# Autodesk Inventor assembly: mearm 期末組合
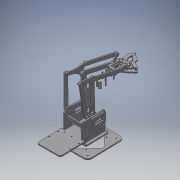
[picture p0: Inventor's stored thumbnail of the model, 180x180]
Saved by Autodesk Inventor 2019 (Build 230136000, 136)
## iProperties
Created: 2022-01-10
Part Number: mearm 期末組合
Material: 一般
Document SubType Name: Assembly
Designer: 10617
Author: 10617
## Documents named in this file (31)
- E:\cad2021\data\tmp\cad2021_hw\downloads\meARM\meARM_Inventor\HW1_mearm零組件\HW1_mearm組合.iam
- E:\cad2021\data\tmp\cad2021_hw\downloads\meARM\meARM_Inventor\HW1_mearm零組件\1.ipt
- E:\cad2021\data\tmp\cad2021_hw\downloads\meARM\meARM_Inventor\HW1_mearm零組件\2.ipt
- E:\cad2021\data\tmp\cad2021_hw\downloads\meARM\meARM_Inventor\HW1_mearm零組件\3.ipt
- E:\cad2021\data\tmp\cad2021_hw\downloads\meARM\meARM_Inventor\HW1_mearm零組件\4.ipt
- E:\cad2021\data\tmp\cad2021_hw\downloads\meARM\meARM_Inventor\HW1_mearm零組件\5.ipt
- E:\cad2021\data\tmp\cad2021_hw\downloads\meARM\meARM_Inventor\HW1_mearm零組件\6.ipt
- E:\cad2021\data\tmp\cad2021_hw\downloads\meARM\meARM_Inventor\HW1_mearm零組件\7.ipt
- E:\cad2021\data\tmp\cad2021_hw\downloads\meARM\meARM_Inventor\HW1_mearm零組件\8.ipt
- E:\cad2021\data\tmp\cad2021_hw\downloads\meARM\meARM_Inventor\HW1_mearm零組件\9.ipt
- E:\cad2021\data\tmp\cad2021_hw\downloads\meARM\meARM_Inventor\HW1_mearm零組件\10.ipt
- E:\cad2021\data\tmp\cad2021_hw\downloads\meARM\meARM_Inventor\HW1_mearm零組件\11.ipt
- E:\cad2021\data\tmp\cad2021_hw\downloads\meARM\meARM_Inventor\HW1_mearm零組件\12.ipt
- E:\cad2021\data\tmp\cad2021_hw\downloads\meARM\meARM_Inventor\HW1_mearm零組件\13.ipt
- E:\cad2021\data\tmp\cad2021_hw\downloads\meARM\meARM_Inventor\HW1_mearm零組件\14.ipt
- E:\cad2021\data\tmp\cad2021_hw\downloads\meARM\meARM_Inventor\HW1_mearm零組件\15.ipt
- E:\cad2021\data\tmp\cad2021_hw\downloads\meARM\meARM_Inventor\HW1_mearm零組件\16.ipt
- E:\cad2021\data\tmp\cad2021_hw\downloads\meARM\meARM_Inventor\HW1_mearm零組件\17.ipt
- E:\cad2021\data\tmp\cad2021_hw\downloads\meARM\meARM_Inventor\HW1_mearm零組件\18.ipt
- E:\cad2021\data\tmp\cad2021_hw\downloads\meARM\meARM_Inventor\HW1_mearm零組件\19.ipt
- E:\cad2021\data\tmp\cad2021_hw\downloads\meARM\meARM_Inventor\HW1_mearm零組件\20.ipt
- E:\cad2021\data\tmp\cad2021_hw\downloads\meARM\meARM_Inventor\HW1_mearm零組件\21.ipt
- E:\cad2021\data\tmp\cad2021_hw\downloads\meARM\meARM_Inventor\HW1_mearm零組件\22.ipt
- E:\cad2021\data\tmp\cad2021_hw\downloads\meARM\meARM_Inventor\HW1_mearm零組件\24.ipt
- E:\cad2021\data\tmp\cad2021_hw\downloads\meARM\meARM_Inventor\HW1_mearm零組件\25.ipt
- E:\cad2021\data\tmp\cad2021_hw\downloads\meARM\meARM_Inventor\HW1_mearm零組件\26.ipt
- E:\cad2021\data\tmp\cad2021_hw\downloads\meARM\meARM_Inventor\HW1_mearm零組件\27.ipt
- E:\cad2021\data\tmp\cad2021_hw\downloads\meARM\meARM_Inventor\HW1_mearm零組件\齒輪.ipt
- E:\cad2021\data\tmp\cad2021_hw\downloads\meARM\meARM_Inventor\HW1_mearm零組件\齒輪2.ipt
- E:\cad2021\data\tmp\cad2021_hw\downloads\meARM\meARM_Inventor\HW1_mearm零組件\23.ipt
- E:\cad2021\data\tmp\cad2021_hw\downloads\meARM\meARM_Inventor\HW1_mearm零組件\軸.ipt
## Components (48 placed, 30 different names)
1. 1:1 — 貼合:30, 貼合:31, 貼合:32, 貼合:42, 貼合:46, 貼合:47
2. 2:1 — 貼合:33, 貼合:34, 貼合:35, 貼合:36, 貼合:37, 貼合:41
3. 3:1 — 貼合:38, 貼合:39, 貼合:44, 貼合:45
4. 4:1 — 貼合:48, 貼合:49, 貼合:70, 貼合:76
5. 5:1 — 貼合:28, 貼合:40, 貼合:79
6. 6:1 — 齊平:1, 貼合:1, 貼合:2, 貼合:3, 角度:2, 齊平:3, 角度:3, 齊平:6, 齊平:7, 角度:6
7. 7:1 — 角度:2, 齊平:3, 齊平:4, 齊平:5
8. 8:1 — 貼合:13, 貼合:14, 齊平:9
9. 9:1 — 貼合:25, 貼合:26, 貼合:27, 齊平:11
10. 10:1 — 貼合:11, 齊平:8, 貼合:12
11. 11:1 — 角度:3, 齊平:6, 齊平:7, 貼合:5, 貼合:6, 貼合:7, 貼合:8, 貼合:9, 貼合:10, 貼合:17, 貼合:19
12. 12:1 — 貼合:30, 貼合:31, 貼合:32, 貼合:33, 貼合:34, 貼合:35
13. 13:1 — 貼合:42, 貼合:44, 貼合:45, 貼合:48, 貼合:49
14. 14:1 — 貼合:8, 貼合:9, 貼合:10, 貼合:15, 貼合:16, 齊平:10, 角度:4, 貼合:18, 貼合:25, 貼合:27
15. 15:1 — 貼合:46, 貼合:47, 貼合:73, 貼合:74
16. 16:1 — 貼合:5, 貼合:6, 貼合:7, 貼合:11, 齊平:8, 貼合:12, 貼合:13, 貼合:14, 齊平:9, 貼合:26, 貼合:38, 貼合:39
17. 17:1 — 貼合:15, 貼合:16, 齊平:10
18. 18:1 — 齊平:12, 齊平:13, 貼合:54, 貼合:55, 貼合:82
19. 19:1 — 貼合:80, 貼合:81, 貼合:82, 貼合:83
20. 20:1 — 貼合:77, 貼合:78, 貼合:79
21. 21:1 — 貼合:17, 角度:4, 貼合:18, 貼合:19, 貼合:36, 貼合:37, 貼合:77, 貼合:78
22. 22:1 — 齊平:1, 貼合:1, 貼合:2, 貼合:3, 齊平:4, 齊平:5, 齊平:11
23. 24:1 — 貼合:51, 貼合:52, 貼合:53, 貼合:54, 貼合:70, 貼合:74, 貼合:76
24. 25:1 — 貼合:63, 貼合:80, 貼合:81, 貼合:84
25. 26:1 — 貼合:55, 貼合:56, 貼合:57, 貼合:67, 貼合:83
26. 27:1 — 貼合:28, 貼合:40, 貼合:41, 貼合:67, 貼合:73
27. 齒輪:1 — 貼合:58, 貼合:60, 貼合:63, 貼合:84
28. 齒輪2:1 — 貼合:59, 貼合:61
29. 23:1 — 齊平:12, 齊平:13, 貼合:51, 貼合:52, 貼合:53, 貼合:56, 貼合:57, 貼合:58, 貼合:59, 貼合:60, 貼合:61, 角度:6
30. 軸:1
31. 軸:2
32. 軸:3
33. 軸:4
34. 軸:5
35. 軸:6
36. 軸:7
37. 軸:8
38. 軸:9
39. 軸:10
40. 軸:11
41. 軸:12
42. 軸:13
43. 軸:14
44. 軸:15
45. 軸:16
46. 軸:17
47. 軸:18
48. 軸:19
## Relationships (82: Mate 66, Flush 12, Angle 4)
- 齊平:1 [Flush] (13 mm): 6:1 ↔ 22:1
- 貼合:1 [Mate]: 6:1 ↔ 22:1
- 貼合:2 [Mate]: 6:1 ↔ 22:1
- 貼合:3 [Mate]: 6:1 ↔ 22:1
- 角度:2 [Angle] (0 deg): 6:1 ↔ 7:1
- 齊平:3 [Flush] (-7.63 mm): 6:1 ↔ 7:1
- 齊平:4 [Flush]: 7:1 ↔ 22:1
- 齊平:5 [Flush]: 7:1 ↔ 22:1
- 角度:3 [Angle] (0 deg): 6:1 ↔ 11:1
- 齊平:6 [Flush] (21.31 mm): 6:1 ↔ 11:1
- 齊平:7 [Flush] (-24.48 mm): 6:1 ↔ 11:1
- 貼合:5 [Mate]: 11:1 ↔ 16:1
- 貼合:6 [Mate]: 11:1 ↔ 16:1
- 貼合:7 [Mate]: 11:1 ↔ 16:1
- 貼合:8 [Mate]: 11:1 ↔ 14:1
- 貼合:9 [Mate]: 11:1 ↔ 14:1
- 貼合:10 [Mate]: 11:1 ↔ 14:1
- 貼合:11 [Mate]: 10:1 ↔ 16:1
- 齊平:8 [Flush]: 10:1 ↔ 16:1
- 貼合:12 [Mate]: 10:1 ↔ 16:1
- 貼合:13 [Mate]: 8:1 ↔ 16:1
- 貼合:14 [Mate]: 8:1 ↔ 16:1
- 齊平:9 [Flush] (-5.37 mm): 8:1 ↔ 16:1
- 貼合:15 [Mate]: 14:1 ↔ 17:1
- 貼合:16 [Mate]: 14:1 ↔ 17:1
- 齊平:10 [Flush] (-5.37 mm): 14:1 ↔ 17:1
- 貼合:17 [Mate]: 11:1 ↔ 21:1
- 角度:4 [Angle] (0 deg): 14:1 ↔ 21:1
- 貼合:18 [Mate] (11.88 mm): 14:1 ↔ 21:1
- 貼合:19 [Mate] (3 mm): 11:1 ↔ 21:1
- 貼合:25 [Mate]: 9:1 ↔ 14:1
- 貼合:26 [Mate]: 9:1 ↔ 16:1
- 貼合:27 [Mate]: 9:1 ↔ 14:1
- 貼合:28 [Mate]: 5:1 ↔ 27:1
- 貼合:30 [Mate]: 1:1 ↔ 12:1
- 貼合:31 [Mate]: 1:1 ↔ 12:1
- 貼合:32 [Mate]: 1:1 ↔ 12:1
- 貼合:33 [Mate]: 2:1 ↔ 12:1
- 貼合:34 [Mate]: 2:1 ↔ 12:1
- 貼合:35 [Mate]: 2:1 ↔ 12:1
- 貼合:36 [Mate]: 2:1 ↔ 21:1
- 貼合:37 [Mate]: 2:1 ↔ 21:1
- 貼合:38 [Mate]: 3:1 ↔ 16:1
- 貼合:39 [Mate]: 3:1 ↔ 16:1
- 貼合:40 [Mate]: 5:1 ↔ 27:1
- 貼合:41 [Mate]: 2:1 ↔ 27:1
- 貼合:42 [Mate]: 1:1 ↔ 13:1
- 貼合:44 [Mate]: 3:1 ↔ 13:1
- 貼合:45 [Mate] (1 mm): 3:1 ↔ 13:1
- 貼合:46 [Mate]: 1:1 ↔ 15:1
- 貼合:47 [Mate]: 1:1 ↔ 15:1
- 貼合:48 [Mate]: 4:1 ↔ 13:1
- 貼合:49 [Mate]: 4:1 ↔ 13:1
- 齊平:11 [Flush] (6.88 mm): 9:1 ↔ 22:1
- 齊平:12 [Flush]: 18:1 ↔ 23:1
- 齊平:13 [Flush]: 18:1 ↔ 23:1
- 貼合:51 [Mate]: 24:1 ↔ 23:1
- 貼合:52 [Mate]: 24:1 ↔ 23:1
- 貼合:53 [Mate]: 24:1 ↔ 23:1
- 貼合:54 [Mate]: 18:1 ↔ 24:1
- 貼合:55 [Mate]: 18:1 ↔ 26:1
- 貼合:56 [Mate]: 26:1 ↔ 23:1
- 貼合:57 [Mate]: 26:1 ↔ 23:1
- 貼合:58 [Mate]: 齒輪:1 ↔ 23:1
- 貼合:59 [Mate]: 齒輪2:1 ↔ 23:1
- 貼合:60 [Mate] (0.2 mm): 齒輪:1 ↔ 23:1
- 貼合:61 [Mate] (0.2 mm): 齒輪2:1 ↔ 23:1
- 貼合:63 [Mate] (0.2 mm): 25:1 ↔ 齒輪:1
- 貼合:67 [Mate]: 26:1 ↔ 27:1
- 貼合:70 [Mate]: 4:1 ↔ 24:1
- 貼合:73 [Mate]: 15:1 ↔ 27:1
- 貼合:74 [Mate]: 15:1 ↔ 24:1
- 角度:6 [Angle] (0 deg): 6:1 ↔ 23:1
- 貼合:76 [Mate]: 4:1 ↔ 24:1
- 貼合:77 [Mate]: 20:1 ↔ 21:1
- 貼合:78 [Mate] (4.4 mm): 20:1 ↔ 21:1
- 貼合:79 [Mate]: 5:1 ↔ 20:1
- 貼合:80 [Mate]: 19:1 ↔ 25:1
- 貼合:81 [Mate] (4.48 mm): 19:1 ↔ 25:1
- 貼合:82 [Mate] (-11 mm): 18:1 ↔ 19:1
- 貼合:83 [Mate] (-12 mm): 19:1 ↔ 26:1
- 貼合:84 [Mate]: 25:1 ↔ 齒輪:1
